# Autodesk Inventor assembly: 2 mm
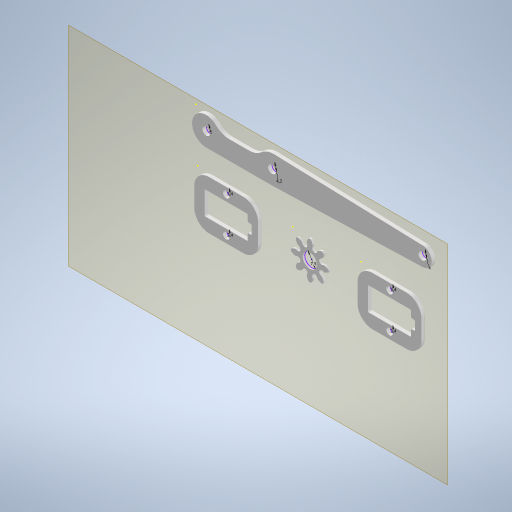
[picture p0: Inventor's stored thumbnail of the model, 512x512]
Saved by Autodesk Inventor 2023 (Build 270158000, 158)
## iProperties
Created: 2023-11-09
Part Number: 2 mm
Document SubType Name: Assembly
Designer: JULIAN
Author: JULIAN
## Documents named in this file (4)
- C:\Users\JULIAN\Desktop\Materias UN\Taller de Ingeniería Electrónica\Modelado cargo bot\DWG\2 mm.iam
- C:\Users\JULIAN\Desktop\Materias UN\Taller de Ingeniería Electrónica\Modelado cargo bot\Modelado\Ajuste servo.ipt
- C:\Users\JULIAN\Desktop\Materias UN\Taller de Ingeniería Electrónica\Modelado cargo bot\Modelado\Brazo horizontal.ipt
- C:\Users\JULIAN\Desktop\Materias UN\Taller de Ingeniería Electrónica\Modelado cargo bot\Modelado\Engrane 2.ipt
## Components (4 placed, 3 different names)
1. Ajuste servo:1 — Coincidencia:1
2. Brazo horizontal:1 — Coincidencia:2
3. Engrane 2:1 — Coincidencia:3
4. Ajuste servo:2 — Coincidencia:4
## Relationships (4: Mate 4)
- Coincidencia:1 [Mate]: Ajuste servo:1
- Coincidencia:2 [Mate]: Brazo horizontal:1
- Coincidencia:3 [Mate]: Engrane 2:1
- Coincidencia:4 [Mate]: Ajuste servo:2
